# Autodesk Inventor assembly: Сборка1
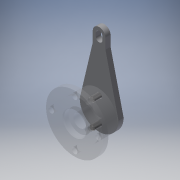
[picture p0: Inventor's stored thumbnail of the model, 180x180]
Saved by Autodesk Inventor 2019 (Build 230136000, 136)
## iProperties
Created: 2020-04-07
Part Number: Сборка1
Material: Типовые
Document SubType Name: Assembly
Designer: Diana
Mass: 349.428 g
Surface Area: 611.26 cm^2
Volume: 314.002 cm^3
Density: 1.11282 g/cm^3
Author: Diana
## Documents named in this file (5)
- C:\Users\Diana\Documents\Inventor\Инж_граф\Сборка\Сборка1.iam
- C:\Users\Diana\Documents\Inventor\Инж_граф\Сборка\Рычаг.ipt
- Рычаг.ipt
- C:\Users\Diana\Documents\Inventor\Инж_граф\Сборка\Фланец.ipt
- C:\Users\Diana\Documents\Inventor\Content Center Files\R2019\ru-RU\GOST 17474-80 (1)\Винт M10-6gx25 ГОСТ 17474-80.ipt
## Components (4 placed, 3 different names)
1. Рычаг:1 — Совмещение:1, Совмещение:2, Совмещение:3, Совмещение:4, Совмещение:5
2. Фланец:1 — Совмещение:1, Совмещение:2, Совмещение:3
3. Винт ГОСТ 17474-80 M10 x 25:1 — Совмещение:4
4. Винт ГОСТ 17474-80 M10 x 25:2 — Совмещение:5
## Relationships (5: Mate 5)
- Совмещение:1 [Mate]: Рычаг:1 ↔ Фланец:1
- Совмещение:2 [Mate]: Рычаг:1 ↔ Фланец:1
- Совмещение:3 [Mate]: Рычаг:1 ↔ Фланец:1
- Совмещение:4 [Mate]: Рычаг:1 ↔ Винт ГОСТ 17474-80 M10 x 25:1
- Совмещение:5 [Mate]: Рычаг:1 ↔ Винт ГОСТ 17474-80 M10 x 25:2
